# Autodesk Inventor assembly: Pigeon 2
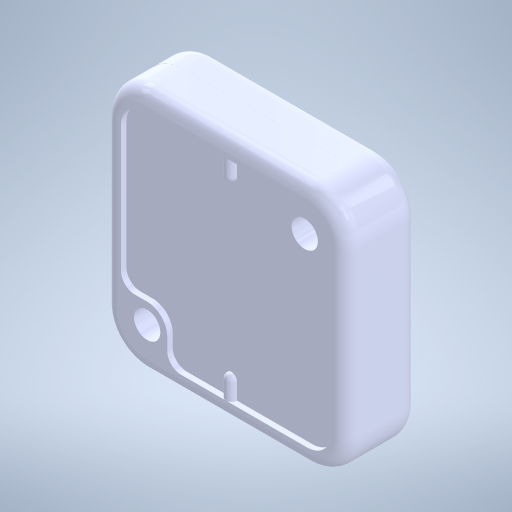
[picture p0: Inventor's stored thumbnail of the model, 512x512]
Saved by Autodesk Inventor 2023.3 (Build 273359000, 359)
## iProperties
Created: 2023-10-13
Part Number: Pigeon 2
Document SubType Name: Assembly
Designer: jackc
Author: jackc
Revision Number: ANY
## Documents named in this file (3)
- D:\.shortcut-targets-by-id\104lhnwPhYvankLacu8RGROV89Bx_24Mg\1939\2_Design\2023-2024\Parts\Electronics\Pigeon\Pigeon 2.iam
- D:\.shortcut-targets-by-id\104lhnwPhYvankLacu8RGROV89Bx_24Mg\1939\2_Design\2023-2024\Parts\Electronics\Pigeon\Bot Housing.ipt
- D:\.shortcut-targets-by-id\104lhnwPhYvankLacu8RGROV89Bx_24Mg\1939\2_Design\2023-2024\Parts\Electronics\Pigeon\Top Housing.ipt
## Components (2 placed, 2 different names)
1. Bot Housing:1 — Mate:1, Mate:2, Mate:3
2. Top Housing:1 — Mate:1, Mate:2, Mate:3
## Relationships (3: Mate 3)
- Mate:1: Bot Housing:1 ↔ Top Housing:1
- Mate:2: Bot Housing:1 ↔ Top Housing:1
- Mate:3: Bot Housing:1 ↔ Top Housing:1
